# Autodesk Inventor assembly: Ensamblaje1
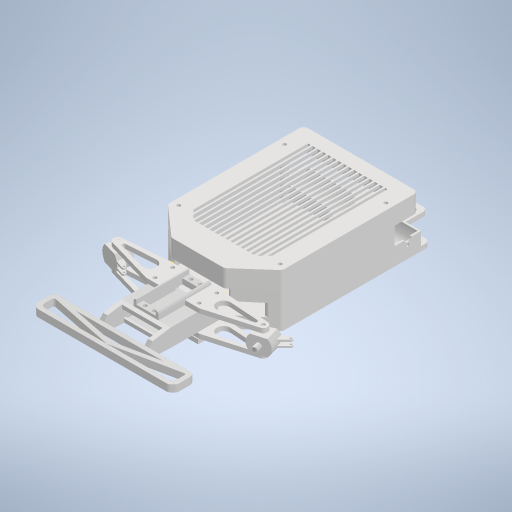
[picture p0: Inventor's stored thumbnail of the model, 512x512]
Saved by Autodesk Inventor 2024.3 (Build 283343000, 343)
## iProperties
Created: 2025-01-30
Part Number: Ensamblaje1
Document SubType Name: Assembly
Designer: Jorge
Author: Jorge
## Documents named in this file (8)
- C:\Users\Jorge\Desktop\Auto Autónomo\Ensamblaje1.iam
- C:\Users\Jorge\Desktop\Auto Autónomo\Pieza1.ipt
- C:\Users\Jorge\Desktop\Auto Autónomo\Pieza3.ipt
- C:\Users\Jorge\Desktop\Auto Autónomo\Pieza4.ipt
- C:\Users\Jorge\Desktop\Auto Autónomo\Pieza5.ipt
- C:\Users\Jorge\Desktop\Auto Autónomo\Pieza6.ipt
- C:\Users\Jorge\Desktop\Auto Autónomo\Pieza7.ipt
- C:\Users\Jorge\Documents\Inventor\Pieza2.ipt
## Components (10 placed, 7 different names)
1. Pieza1:1 — Rígido:2, De rotación:1, Rígido:3, De rotación:3
2. Pieza3:1 — Rígido:2, Rígido:5
3. Pieza3:2 — De rotación:1, De rotación:4
4. Pieza4:1 — Rígido:3, Rígido:4
5. Pieza5:1 — Rígido:4
6. Pieza7:1 — De rotación:3, De rotación:6
7. Pieza6:1 — De rotación:6
8. Pieza6:2 — De rotación:5
9. Pieza7:2 — De rotación:4, De rotación:5
10. Pieza2:2 — Rígido:5
## Relationships (9: RevoluteJoint 5, WeldJoint 4)
- Rígido:2 [WeldJoint] (20 mm): Pieza1:1 ↔ Pieza3:1
- De rotación:1 [RevoluteJoint] (20 mm): Pieza1:1 ↔ Pieza3:2
- Rígido:3 [WeldJoint]: Pieza1:1 ↔ Pieza4:1
- Rígido:4 [WeldJoint]: Pieza4:1 ↔ Pieza5:1
- De rotación:3 [RevoluteJoint]: Pieza1:1 ↔ Pieza7:1
- De rotación:4 [RevoluteJoint]: Pieza3:2 ↔ Pieza7:2
- Rígido:5 [WeldJoint]: Pieza3:1 ↔ Pieza2:2
- De rotación:5 [RevoluteJoint]: Pieza6:2 ↔ Pieza7:2
- De rotación:6 [RevoluteJoint]: Pieza7:1 ↔ Pieza6:1
